# Autodesk Inventor assembly: printer
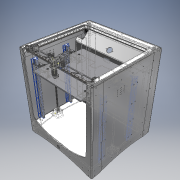
[picture p0: Inventor's stored thumbnail of the model, 180x180]
Saved by Autodesk Inventor 2017 (Build 210142000, 142)
## iProperties
Created: 2016-06-10
Part Number: printer
Document SubType Name: Assembly
Designer: brent
Author: brent
## Documents named in this file (15)
- C:\Users\yibre\OneDrive\personal\printer_mechanical\printer.iam
- C:\Users\yibre\OneDrive\personal\printer_mechanical\frame.ipt
- C:\Users\yibre\OneDrive\personal\printer_mechanical\x_gantry.iam
- C:\Users\yibre\OneDrive\personal\printer_mechanical\offtheshelf\linear_stepper_350mm.ipt
- C:\Users\yibre\OneDrive\personal\printer_mechanical\offtheshelf\sbr12_350mm.ipt
- C:\Users\yibre\OneDrive\personal\printer_mechanical\offtheshelf\nema17_40mm.ipt
- C:\Users\yibre\OneDrive\personal\printer_mechanical\offtheshelf\20t_gt2_6mm_pulley.ipt
- C:\Users\yibre\OneDrive\personal\printer_mechanical\offtheshelf\mgn9_350mm.ipt
- C:\Users\yibre\OneDrive\personal\printer_mechanical\offtheshelf\20t_gt2_6mm_idler.ipt
- C:\Users\yibre\OneDrive\personal\printer_mechanical\z_assembly.iam
- C:\Users\yibre\OneDrive\personal\printer_mechanical\offtheshelf\16mm_switch.ipt
- C:\Users\yibre\OneDrive\personal\printer_mechanical\printer\Design Accelerator\Bolted Connection1.iam
- C:\Users\yibre\OneDrive\personal\printer_mechanical\spacers\m5_spacer.ipt
- C:\Users\yibre\OneDrive\personal\printer_mechanical\printer\Design Accelerator\Bolted Connection2.iam
- C:\Users\yibre\OneDrive\personal\printer_mechanical\printer\Design Accelerator\Bolted Connection3.iam
## Components (23 placed, 12 different names)
1. frame:1 — Mate:2, Mate:3, Mate:4, Mate:5, Mate:6, Mate:7, Mate:9, Mate:12, Mate:16, Mate:19, Mate:20, Mate:21, Mate:22, Mate:23, Mate:25, Mate:26, Mate:29, Mate:32, Mate:33, Mate:34, Mate:35, Mate:36, Mate:37, Mate:38, Mate:39, Mate:40, Mate:44, Mate:45, Mate:48, Mate:54, Mate:55, Mate:56, Mate:59, Mate:60, Mate:61, Mate:62
2. x_gantry:1 [sub-assembly] — Mate:2, Mate:3, Mate:41
3. linear_stepper_350mm:1 — Mate:4, Mate:7
4. linear_stepper_350mm:2 — Mate:5, Mate:6
5. sbr12_350mm:1 — Mate:9, Mate:57, Mate:60
6. sbr12_350mm:2 — Mate:16, Mate:42, Mate:54, Mate:55
7. sbr12_350mm:3 — Mate:19, Mate:43, Mate:56
8. sbr12_350mm:4 — Mate:12, Mate:58, Mate:59
9. nema17_40mm:1 — Mate:22, Mate:23, Mate:27
10. nema17_40mm:2 — Mate:20, Mate:21, Mate:24, Mate:26
11. 20t_gt2_6mm_pulley:1 — Mate:24, Mate:25
12. 20t_gt2_6mm_pulley:2 — Mate:27, Mate:41
13. mgn9_350mm:1 — Mate:29, Mate:35, Mate:36
14. mgn9_350mm:2 — Mate:32, Mate:33, Mate:34
15. 20t_gt2_6mm_idler:1 — Mate:39, Mate:40, Mate:46, Mate:47
16. 20t_gt2_6mm_idler:2 — Mate:37, Mate:38, Mate:50, Mate:51
17. z_assembly:1 [sub-assembly] — Mate:42, Mate:43, Mate:57, Mate:58
18. 16mm_switch:1 — Mate:44, Mate:45
19. Bolted Connection:1 [sub-assembly] — Mate:46, Mate:47, Mate:49
20. m5_spacer:1 — Mate:48, Mate:49
21. m5_spacer:2 — Mate:50, Mate:51, Mate:52, Mate:53
22. Bolted Connection:2 [sub-assembly] — Mate:52, Mate:53
23. Bolted Connection:3 [sub-assembly] — Mate:61, Mate:62
## Relationships (50: Mate 50)
- Mate:2 (5 mm): frame:1 ↔ x_gantry:1
- Mate:3 (6.5 mm): frame:1 ↔ x_gantry:1
- Mate:4: frame:1 ↔ linear_stepper_350mm:1
- Mate:5: frame:1 ↔ linear_stepper_350mm:2
- Mate:6: frame:1 ↔ linear_stepper_350mm:2
- Mate:7: frame:1 ↔ linear_stepper_350mm:1
- Mate:9: frame:1 ↔ sbr12_350mm:1
- Mate:12: frame:1 ↔ sbr12_350mm:4
- Mate:16: frame:1 ↔ sbr12_350mm:2
- Mate:19: frame:1 ↔ sbr12_350mm:3
- Mate:20: frame:1 ↔ nema17_40mm:2
- Mate:21: frame:1 ↔ nema17_40mm:2
- Mate:22: frame:1 ↔ nema17_40mm:1
- Mate:23: frame:1 ↔ nema17_40mm:1
- Mate:24: nema17_40mm:2 ↔ 20t_gt2_6mm_pulley:1
- Mate:25: frame:1 ↔ 20t_gt2_6mm_pulley:1
- Mate:26: frame:1 ↔ nema17_40mm:2
- Mate:27: nema17_40mm:1 ↔ 20t_gt2_6mm_pulley:2
- Mate:29: frame:1 ↔ mgn9_350mm:1
- Mate:32: frame:1 ↔ mgn9_350mm:2
- Mate:33: frame:1 ↔ mgn9_350mm:2
- Mate:34: frame:1 ↔ mgn9_350mm:2
- Mate:35: frame:1 ↔ mgn9_350mm:1
- Mate:36: frame:1 ↔ mgn9_350mm:1
- Mate:37: frame:1 ↔ 20t_gt2_6mm_idler:2
- Mate:38: frame:1 ↔ 20t_gt2_6mm_idler:2
- Mate:39: frame:1 ↔ 20t_gt2_6mm_idler:1
- Mate:40: frame:1 ↔ 20t_gt2_6mm_idler:1
- Mate:41: x_gantry:1 ↔ 20t_gt2_6mm_pulley:2
- Mate:42: sbr12_350mm:2 ↔ z_assembly:1
- Mate:43: sbr12_350mm:3 ↔ z_assembly:1
- Mate:44: frame:1 ↔ 16mm_switch:1
- Mate:45: frame:1 ↔ 16mm_switch:1
- Mate:46: 20t_gt2_6mm_idler:1 ↔ Bolted Connection:1
- Mate:47: 20t_gt2_6mm_idler:1 ↔ Bolted Connection:1
- Mate:48: frame:1 ↔ m5_spacer:1
- Mate:49: Bolted Connection:1 ↔ m5_spacer:1
- Mate:50: 20t_gt2_6mm_idler:2 ↔ m5_spacer:2
- Mate:51: 20t_gt2_6mm_idler:2 ↔ m5_spacer:2
- Mate:52: m5_spacer:2 ↔ Bolted Connection:2
- Mate:53: m5_spacer:2 ↔ Bolted Connection:2
- Mate:54: frame:1 ↔ sbr12_350mm:2
- Mate:55: frame:1 ↔ sbr12_350mm:2
- Mate:56: frame:1 ↔ sbr12_350mm:3
- Mate:57: sbr12_350mm:1 ↔ z_assembly:1
- Mate:58: sbr12_350mm:4 ↔ z_assembly:1
- Mate:59: frame:1 ↔ sbr12_350mm:4
- Mate:60: frame:1 ↔ sbr12_350mm:1
- Mate:61: frame:1 ↔ Bolted Connection:3
- Mate:62: frame:1 ↔ Bolted Connection:3
